# Autodesk Inventor assembly: Собранная Мясорубка
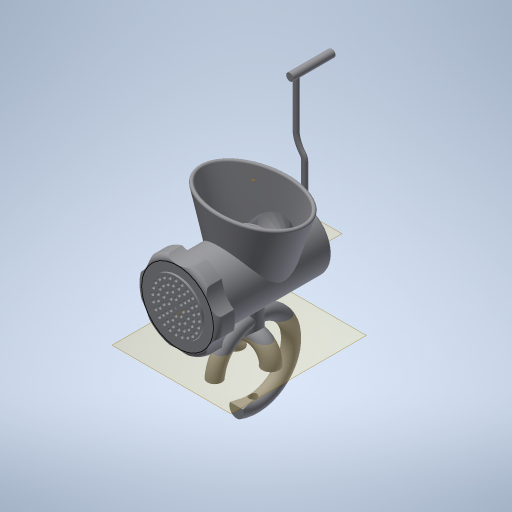
[picture p0: Inventor's stored thumbnail of the model, 512x512]
Saved by Autodesk Inventor 2023.2 (Build 272271030, 271C)
## iProperties
Created: 2023-07-20
Part Number: Собранная Мясорубка
Document SubType Name: Assembly
Designer: 1.507-10
Author: 1.507-10
## Documents named in this file (7)
- C:\Users\Personal Computer\Desktop\SKGMI\MyPractice\Инвентор\лабораторная работа №5\собранная мясорубка.iam
- C:\Users\Personal Computer\Desktop\SKGMI\MyPractice\Инвентор\лабораторная работа №5\Крышка.ipt
- C:\Users\Personal Computer\Desktop\SKGMI\MyPractice\Инвентор\лабораторная работа №5\Матрица.ipt
- C:\Users\Personal Computer\Desktop\SKGMI\MyPractice\Инвентор\лабораторная работа №5\Нож.ipt
- C:\Users\Personal Computer\Desktop\SKGMI\MyPractice\Инвентор\лабораторная работа №5\Рукоять.ipt
- C:\Users\Personal Computer\Desktop\SKGMI\MyPractice\Инвентор\лабораторная работа №5\Шнек.ipt
- C:\Users\Personal Computer\Desktop\SKGMI\MyPractice\Инвентор\лабораторная работа №5\Корпус.ipt
## Components (6 placed, 6 different names)
1. Корпус:1 — Вращательный:1, Вращательный:3, Flush:1
2. Крышка:1 — Вращательный:2, Flush:1
3. Матрица:1 — Вращательный:2, Жесткий:2
4. Нож:1 — Жесткий:1
5. Рукоять:1 — Вращательный:3
6. Шнек:1 — Жесткий:1, Вращательный:1, Жесткий:2
## Relationships (6: RevoluteJoint 3, WeldJoint 2, Flush 1)
- Жесткий:1 [WeldJoint]: Нож:1 ↔ Шнек:1
- Вращательный:1 [RevoluteJoint]: Корпус:1 ↔ Шнек:1
- Вращательный:2 [RevoluteJoint]: Крышка:1 ↔ Матрица:1
- Жесткий:2 [WeldJoint]: Матрица:1 ↔ Шнек:1
- Вращательный:3 [RevoluteJoint]: Корпус:1 ↔ Рукоять:1
- Flush:1 (100 mm): Корпус:1 ↔ Крышка:1
